# Autodesk Inventor assembly: 200-40-BOGIE-CONNECTOR-REINFORCEMENT-01
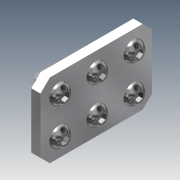
[picture p0: Inventor's stored thumbnail of the model, 180x180]
Saved by Autodesk Inventor 2018.2 (Build 222227000, 227)
## iProperties
Manager: feesmrt
Company: FRANCOR
Part Number: 200-40-BOGIE-CONNECTOR-REINFORCEMENT-01
Project: Rescue Robot
Cost Center: -
Material: Generisch
Document SubType Name: Assembly
Designer: feesmrt
Engineer: feesmrt
Authority: feesmrt
Description: Bogie Connector Verstärkung
Stock Number: 200-40-BOGIE-CONNECTOR-REINFORCEMENT-01
Subject: Rescue Robot
Author: feesmrt
Revision Number: 1
Title: Bogie Connector Verstärkung
## Documents named in this file (4)
- D:\Programmierung\FRANC0R\CAD\02-Rocker-Bogie-Robot\200-ROCKER-BOGIE\200-40-BOGIE-CONNECTOR\200-40-BOGIE-CONNECTOR-REINFORCEMENT-01.iam
- D:\Programmierung\FRANC0R\CAD\02-Rocker-Bogie-Robot\200-ROCKER-BOGIE\200-40-BOGIE-CONNECTOR\200-40-BOGIE-CONNECTOR-06.ipt
- D:\Programmierung\FRANC0R\CAD\02-Rocker-Bogie-Robot\900-COMPONENTS\900-50-PROFILES\900-50-PROFILES-CONN-N6xM5.ipt
- D:\Programmierung\FRANC0R\CAD\02-Rocker-Bogie-Robot\900-COMPONENTS\900-40-SCREWS\900-40-SCREWS-ISO7830_M6x10.ipt
## Components (13 placed, 3 different names)
1. 200-40-BOGIE-CONNECTOR-06:1 — Passend:1, Passend:2, Passend:3, Passend:4, Passend:5, Passend:6, Passend:7, Passend:8, Passend:9, Passend:10, Passend:11, Passend:12, Winkel:1, Winkel:2, Winkel:3, Winkel:4, Winkel:5, Winkel:6, Passend:13, Passend:14, Passend:15, Passend:16, Passend:17, Passend:18, Passend:19, Passend:20, Passend:21, Passend:22, Passend:23, Passend:24
2. 900-50-PROFILES-CONN-N6xM5:1 — Passend:1, Passend:7, Winkel:5
3. 900-50-PROFILES-CONN-N6xM5:2 — Passend:2, Passend:8, Winkel:6
4. 900-50-PROFILES-CONN-N6xM5:3 — Passend:3, Passend:9, Winkel:1
5. 900-50-PROFILES-CONN-N6xM5:4 — Passend:4, Passend:10, Winkel:2
6. 900-50-PROFILES-CONN-N6xM5:5 — Passend:5, Passend:11, Winkel:3
7. 900-50-PROFILES-CONN-N6xM5:6 — Passend:6, Passend:12, Winkel:4
8. 900-40-SCREWS-ISO7830_M6x10:1 — Passend:13, Passend:19
9. 900-40-SCREWS-ISO7830_M6x10:2 — Passend:14, Passend:20
10. 900-40-SCREWS-ISO7830_M6x10:3 — Passend:15, Passend:21
11. 900-40-SCREWS-ISO7830_M6x10:4 — Passend:16, Passend:22
12. 900-40-SCREWS-ISO7830_M6x10:5 — Passend:17, Passend:24
13. 900-40-SCREWS-ISO7830_M6x10:6 — Passend:18, Passend:23
## Relationships (30: Mate 24, Angle 6)
- Passend:1 [Mate]: 200-40-BOGIE-CONNECTOR-06:1 ↔ 900-50-PROFILES-CONN-N6xM5:1
- Passend:2 [Mate]: 200-40-BOGIE-CONNECTOR-06:1 ↔ 900-50-PROFILES-CONN-N6xM5:2
- Passend:3 [Mate]: 200-40-BOGIE-CONNECTOR-06:1 ↔ 900-50-PROFILES-CONN-N6xM5:3
- Passend:4 [Mate]: 200-40-BOGIE-CONNECTOR-06:1 ↔ 900-50-PROFILES-CONN-N6xM5:4
- Passend:5 [Mate]: 200-40-BOGIE-CONNECTOR-06:1 ↔ 900-50-PROFILES-CONN-N6xM5:5
- Passend:6 [Mate]: 200-40-BOGIE-CONNECTOR-06:1 ↔ 900-50-PROFILES-CONN-N6xM5:6
- Passend:7 [Mate] (1.5 mm): 200-40-BOGIE-CONNECTOR-06:1 ↔ 900-50-PROFILES-CONN-N6xM5:1
- Passend:8 [Mate] (1.5 mm): 200-40-BOGIE-CONNECTOR-06:1 ↔ 900-50-PROFILES-CONN-N6xM5:2
- Passend:9 [Mate] (1.5 mm): 200-40-BOGIE-CONNECTOR-06:1 ↔ 900-50-PROFILES-CONN-N6xM5:3
- Passend:10 [Mate] (1.5 mm): 200-40-BOGIE-CONNECTOR-06:1 ↔ 900-50-PROFILES-CONN-N6xM5:4
- Passend:11 [Mate] (1.5 mm): 200-40-BOGIE-CONNECTOR-06:1 ↔ 900-50-PROFILES-CONN-N6xM5:5
- Passend:12 [Mate] (1.5 mm): 200-40-BOGIE-CONNECTOR-06:1 ↔ 900-50-PROFILES-CONN-N6xM5:6
- Winkel:1 [Angle] (0 deg): 200-40-BOGIE-CONNECTOR-06:1 ↔ 900-50-PROFILES-CONN-N6xM5:3
- Winkel:2 [Angle] (0 deg): 200-40-BOGIE-CONNECTOR-06:1 ↔ 900-50-PROFILES-CONN-N6xM5:4
- Winkel:3 [Angle] (0 deg): 200-40-BOGIE-CONNECTOR-06:1 ↔ 900-50-PROFILES-CONN-N6xM5:5
- Winkel:4 [Angle] (0 deg): 200-40-BOGIE-CONNECTOR-06:1 ↔ 900-50-PROFILES-CONN-N6xM5:6
- Winkel:5 [Angle] (0 deg): 200-40-BOGIE-CONNECTOR-06:1 ↔ 900-50-PROFILES-CONN-N6xM5:1
- Winkel:6 [Angle] (0 deg): 200-40-BOGIE-CONNECTOR-06:1 ↔ 900-50-PROFILES-CONN-N6xM5:2
- Passend:13 [Mate]: 200-40-BOGIE-CONNECTOR-06:1 ↔ 900-40-SCREWS-ISO7830_M6x10:1
- Passend:14 [Mate]: 200-40-BOGIE-CONNECTOR-06:1 ↔ 900-40-SCREWS-ISO7830_M6x10:2
- Passend:15 [Mate]: 200-40-BOGIE-CONNECTOR-06:1 ↔ 900-40-SCREWS-ISO7830_M6x10:3
- Passend:16 [Mate]: 200-40-BOGIE-CONNECTOR-06:1 ↔ 900-40-SCREWS-ISO7830_M6x10:4
- Passend:17 [Mate]: 200-40-BOGIE-CONNECTOR-06:1 ↔ 900-40-SCREWS-ISO7830_M6x10:5
- Passend:18 [Mate]: 200-40-BOGIE-CONNECTOR-06:1 ↔ 900-40-SCREWS-ISO7830_M6x10:6
- Passend:19 [Mate]: 200-40-BOGIE-CONNECTOR-06:1 ↔ 900-40-SCREWS-ISO7830_M6x10:1
- Passend:20 [Mate]: 200-40-BOGIE-CONNECTOR-06:1 ↔ 900-40-SCREWS-ISO7830_M6x10:2
- Passend:21 [Mate]: 200-40-BOGIE-CONNECTOR-06:1 ↔ 900-40-SCREWS-ISO7830_M6x10:3
- Passend:22 [Mate]: 200-40-BOGIE-CONNECTOR-06:1 ↔ 900-40-SCREWS-ISO7830_M6x10:4
- Passend:23 [Mate]: 200-40-BOGIE-CONNECTOR-06:1 ↔ 900-40-SCREWS-ISO7830_M6x10:6
- Passend:24 [Mate]: 200-40-BOGIE-CONNECTOR-06:1 ↔ 900-40-SCREWS-ISO7830_M6x10:5
